# Autodesk Inventor assembly: V1
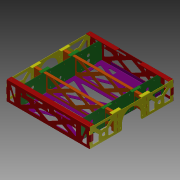
[picture p0: Inventor's stored thumbnail of the model, 180x180]
Saved by Autodesk Inventor 2014 (Build 180170000, 170)
## iProperties
Created: 2014-01-06
Part Number: V1
Document SubType Name: Weldment
Designer: Alex
Weld Material: Welded Aluminum-6061
Author: Alex
## Documents named in this file (8)
- C:\Users\Alex\Documents\Inventor\FRC\V2\Frc Chassis 2014\V1.iam
- C:\Users\Alex\Documents\Inventor\FRC\V2\Frc Chassis 2014\Front.ipt
- C:\Users\Alex\Documents\Inventor\FRC\V2\Frc Chassis 2014\Outer_Side.ipt
- C:\Users\Alex\Documents\Inventor\FRC\V2\Frc Chassis 2014\InnerSide.ipt
- C:\Users\Alex\Documents\Inventor\FRC\V2\Frc Chassis 2014\Brace.ipt
- C:\Users\Alex\Documents\Inventor\FRC\V2\Frc Chassis 2014\Base.ipt
- C:\Users\Alex\Documents\Inventor\FRC\V2\Frc Chassis 2014\Back.ipt
- C:\Users\Alex\Documents\Inventor\FRC\V1\battery.ipt
## Components (10 placed, 7 different names)
1. Outer_Side:1 — Flush:6, Flush:10, Flush:12, Flush:16, Flush:18
2. Outer_Side:2 — Mate:1, Flush:7, Mate:13, Rigid:1
3. InnerSide:2 — Mate:7, Mate:13, Flush:20
4. Brace:1 — Flush:16, Mate:31
5. Brace:2 — Mate:9, Flush:18, Mate:28, Mate:32
6. Base:1 — Flush:19, Mate:33, Mate:34, Flush:20
7. Back:1 — Rigid:1, Mate:33
8. InnerSide:3 — Mate:28, Mate:31, Mate:32, Flush:19, Mate:36
9. Front:1 — Mate:1, Flush:6, Flush:7, Flush:10, Flush:12, Mate:7, Mate:9
10. battery:1 — Mate:34, Mate:36
## Relationships (19: Mate 10, Flush 8, WeldJoint 1)
- Mate:1: Outer_Side:2 ↔ Front:1
- Flush:6: Outer_Side:1 ↔ Front:1
- Flush:7: Outer_Side:2 ↔ Front:1
- Flush:10: Outer_Side:1 ↔ Front:1
- Flush:12: Outer_Side:1 ↔ Front:1
- Mate:7: InnerSide:2 ↔ Front:1
- Flush:16: Outer_Side:1 ↔ Brace:1
- Mate:9 (-228.6 mm): Brace:2 ↔ Front:1
- Flush:18: Outer_Side:1 ↔ Brace:2
- Mate:13 (-101.6 mm): Outer_Side:2 ↔ InnerSide:2
- Rigid:1 [WeldJoint]: Outer_Side:2 ↔ Back:1
- Mate:28: Brace:2 ↔ InnerSide:3
- Mate:31: Brace:1 ↔ InnerSide:3
- Mate:32: Brace:2 ↔ InnerSide:3
- Flush:19: Base:1 ↔ InnerSide:3
- Mate:33: Base:1 ↔ Back:1
- Mate:34: Base:1 ↔ battery:1
- Mate:36 (152.527 mm): InnerSide:3 ↔ battery:1
- Flush:20: InnerSide:2 ↔ Base:1
